# Autodesk Inventor assembly: PipetteSystem
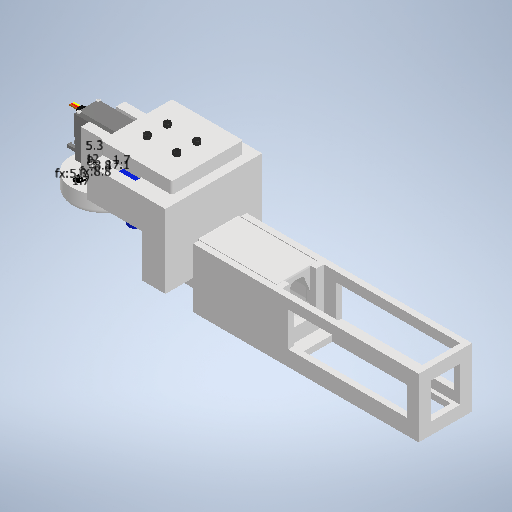
[picture p0: Inventor's stored thumbnail of the model, 512x512]
Saved by Autodesk Inventor 2025.1 (Build 291241000, 241)
## iProperties
Created: 2024-11-13
Part Number: PipetteSystem
Document SubType Name: Assembly
Designer: 13156
Author: 13156
## Documents named in this file (12)
- C:\Users\13156\OneDrive - Binghamton University\Documents\GitHub\Perovskite-Automated-Synthesis-System\CAD\Pipette\PipetteSystem.iam
- C:\Users\13156\OneDrive - Binghamton University\Documents\GitHub\Perovskite-Automated-Synthesis-System\CAD\Pipette\PipetteStand.ipt
- C:\Users\13156\OneDrive - Binghamton University\Documents\GitHub\Perovskite-Automated-Synthesis-System\CAD\Pipette\PipetteSleeveFullLength.ipt
- C:\Users\13156\OneDrive - Binghamton University\Documents\GitHub\Perovskite-Automated-Synthesis-System\CAD\Pipette\HolderMod.ipt
- C:\Users\13156\OneDrive - Binghamton University\Documents\GitHub\Perovskite-Automated-Synthesis-System\CAD\Non 3D Printed Parts\Motors and Servos\SG90 Servo.ipt
- C:\Users\13156\OneDrive - Binghamton University\Documents\GitHub\Perovskite-Automated-Synthesis-System\CAD\Non 3D Printed Parts\Motors and Servos\Servo MG996R.ipt
- C:\Users\13156\OneDrive - Binghamton University\Documents\GitHub\Perovskite-Automated-Synthesis-System\CAD\Pipette\Cam.ipt
- C:\Users\13156\OneDrive - Binghamton University\Documents\GitHub\Perovskite-Automated-Synthesis-System\CAD\Non 3D Printed Parts\Motors and Servos\MG996 2 Arm Pad.ipt
- C:\Users\13156\OneDrive - Binghamton University\Documents\GitHub\Perovskite-Automated-Synthesis-System\CAD\Pipette\Mount.ipt
- C:\Users\13156\OneDrive - Binghamton University\Documents\GitHub\Perovskite-Automated-Synthesis-System\CAD\Non 3D Printed Parts\Screws\M3x6.ipt
- C:\Users\13156\OneDrive - Binghamton University\Documents\GitHub\Perovskite-Automated-Synthesis-System\CAD\Non 3D Printed Parts\Screws\M3x12.ipt
- C:\Users\13156\OneDrive - Binghamton University\Documents\GitHub\Perovskite-Automated-Synthesis-System\CAD\Pipette\GrabberArm.ipt
## Components (18 placed, 11 different names)
1. PipetteStand:1 — Mate:1, Mate:2, Mate:3, Mate:4, Mate:5, Mate:6
2. PipetteSleeveFullLength:1 — Mate:4, Mate:5, Mate:6, Mate:7, Mate:8, Transitional:1, Flush:1
3. HolderMod:1 — Mate:7, Mate:8, Transitional:1, Flush:1, Mate:9, Mate:10, Mate:11, Mate:12, Mate:13, Mate:14, Mate:15, Mate:16, Mate:17, Mate:21, Mate:22, Mate:23, Mate:24, Mate:25, Mate:26, Mate:27, Mate:28, Mate:29, Mate:38, Mate:39, Mate:40, Mate:42, Mate:45, Mate:46, Mate:47
4. SG90 Servo:1 — Mate:9, Mate:10, Mate:11, Mate:38, Mate:39, Mate:40, Mate:42, Mate:43, Flush:3, Mate:45, Mate:46, Mate:47
5. SG90 Servo:2 — Mate:12, Mate:13, Mate:14, Mate:15
6. Servo MG996R:1 — Mate:16, Mate:17, Mate:18, Mate:19
7. Cam:1 — Mate:20, Flush:2
8. MG996 2 Arm Pad:1 — Mate:18, Mate:19, Mate:20, Flush:2
9. Mount:1 — Mate:21, Mate:22, Mate:30, Mate:31, Mate:32, Mate:33, Mate:34, Mate:35, Mate:36, Mate:37
10. M3x6:1 — Mate:23, Mate:24
11. M3x6:2 — Mate:25
12. M3x6:3 — Mate:26, Mate:27
13. M3x6:4 — Mate:28, Mate:29
14. M3x12:1 — Mate:30, Mate:31
15. M3x12:2 — Mate:32, Mate:33
16. M3x12:3 — Mate:34, Mate:35
17. M3x12:4 — Mate:36, Mate:37
18. GrabberArm:1 — Mate:43, Flush:3
## Relationships (49: Mate 45, Flush 3, Transitional 1)
- Mate:1: PipetteStand:1
- Mate:2: PipetteStand:1
- Mate:3: PipetteStand:1
- Mate:4: PipetteStand:1 ↔ PipetteSleeveFullLength:1
- Mate:5: PipetteStand:1 ↔ PipetteSleeveFullLength:1
- Mate:6: PipetteStand:1 ↔ PipetteSleeveFullLength:1
- Mate:7: PipetteSleeveFullLength:1 ↔ HolderMod:1
- Mate:8: PipetteSleeveFullLength:1 ↔ HolderMod:1
- Transitional:1: PipetteSleeveFullLength:1 ↔ HolderMod:1
- Flush:1: PipetteSleeveFullLength:1 ↔ HolderMod:1
- Mate:9: HolderMod:1 ↔ SG90 Servo:1
- Mate:10: HolderMod:1 ↔ SG90 Servo:1
- Mate:11: HolderMod:1 ↔ SG90 Servo:1
- Mate:12: HolderMod:1 ↔ SG90 Servo:2
- Mate:13: HolderMod:1 ↔ SG90 Servo:2
- Mate:14: HolderMod:1 ↔ SG90 Servo:2
- Mate:15: HolderMod:1 ↔ SG90 Servo:2
- Mate:16: HolderMod:1 ↔ Servo MG996R:1
- Mate:17: HolderMod:1 ↔ Servo MG996R:1
- Mate:18 (0.1 mm): Servo MG996R:1 ↔ MG996 2 Arm Pad:1
- Mate:19: Servo MG996R:1 ↔ MG996 2 Arm Pad:1
- Mate:20: Cam:1 ↔ MG996 2 Arm Pad:1
- Flush:2: Cam:1 ↔ MG996 2 Arm Pad:1
- Mate:21: HolderMod:1 ↔ Mount:1
- Mate:22: HolderMod:1 ↔ Mount:1
- Mate:23: HolderMod:1 ↔ M3x6:1
- Mate:24: HolderMod:1 ↔ M3x6:1
- Mate:25: HolderMod:1 ↔ M3x6:2
- Mate:26: HolderMod:1 ↔ M3x6:3
- Mate:27: HolderMod:1 ↔ M3x6:3
- Mate:28: HolderMod:1 ↔ M3x6:4
- Mate:29: HolderMod:1 ↔ M3x6:4
- Mate:30: Mount:1 ↔ M3x12:1
- Mate:31: Mount:1 ↔ M3x12:1
- Mate:32: Mount:1 ↔ M3x12:2
- Mate:33: Mount:1 ↔ M3x12:2
- Mate:34: Mount:1 ↔ M3x12:3
- Mate:35: Mount:1 ↔ M3x12:3
- Mate:36: Mount:1 ↔ M3x12:4
- Mate:37: Mount:1 ↔ M3x12:4
- Mate:38: HolderMod:1 ↔ SG90 Servo:1
- Mate:39: HolderMod:1 ↔ SG90 Servo:1
- Mate:40: HolderMod:1 ↔ SG90 Servo:1
- Mate:42: HolderMod:1 ↔ SG90 Servo:1
- Mate:43: SG90 Servo:1 ↔ GrabberArm:1
- Flush:3 (0.1 mm): SG90 Servo:1 ↔ GrabberArm:1
- Mate:45: HolderMod:1 ↔ SG90 Servo:1
- Mate:46: HolderMod:1 ↔ SG90 Servo:1
- Mate:47: HolderMod:1 ↔ SG90 Servo:1
